# Autodesk Inventor assembly: Sestava1
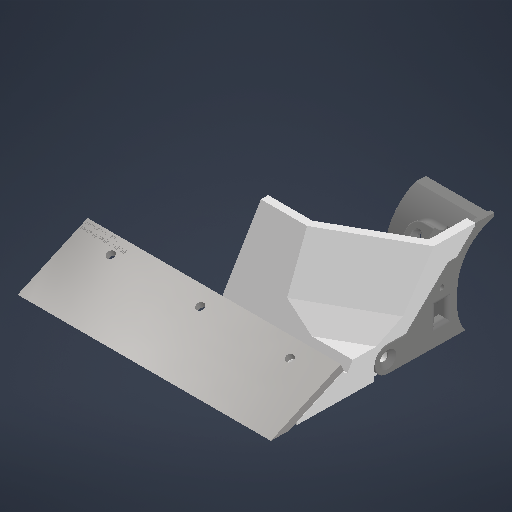
[picture p0: Inventor's stored thumbnail of the model, 512x512]
Saved by Autodesk Inventor 2027 (Build 310192000, 192)
## iProperties
Created: 2026-09-18
Part Number: Sestava1
Document SubType Name: Assembly
Designer: Vadim
Author: Vadim
## Documents named in this file (4)
- C:\Users\Vadim\GitHub\NeoSumec\NeoSumec-MiniSumo-MECH\_MK-1_\Models\Sestava1.iam
- C:\Users\Vadim\GitHub\NeoSumec\NeoSumec-MiniSumo-MECH\_MK-1_\Models\3D_Print\BodyMain.ipt
- C:\Users\Vadim\GitHub\NeoSumec\NeoSumec-MiniSumo-MECH\_MK-1_\Models\3D_Print\BodyFront.ipt
- C:\Users\Vadim\GitHub\NeoSumec\NeoSumec-MiniSumo-MECH\_MK-1_\Models\Metal\Knife.ipt
## Components (3 placed, 3 different names)
1. BodyMain:1 — Proti sobě:1, Proti sobě:2
2. BodyFront:1 — Proti sobě:1, Proti sobě:2, Proti sobě:3, Proti sobě:4, Proti sobě:5
3. Knife:1 — Proti sobě:3, Proti sobě:4, Proti sobě:5
## Relationships (5: Mate 5)
- Proti sobě:1 [Mate]: BodyMain:1 ↔ BodyFront:1
- Proti sobě:2 [Mate] (0.1 mm): BodyMain:1 ↔ BodyFront:1
- Proti sobě:3 [Mate]: BodyFront:1 ↔ Knife:1
- Proti sobě:4 [Mate]: BodyFront:1 ↔ Knife:1
- Proti sobě:5 [Mate]: BodyFront:1 ↔ Knife:1
